# Autodesk Inventor assembly: ECE477
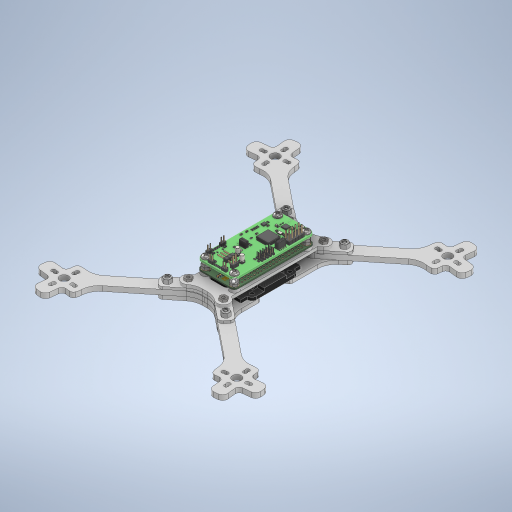
[picture p0: Inventor's stored thumbnail of the model, 512x512]
Saved by Autodesk Inventor 2023 (Build 270158000, 158)
## iProperties
Created: 2022-11-05
Part Number: ECE477
Document SubType Name: Assembly
Designer: mjlangfo
Author: mjlangfo
## Documents named in this file (9)
- \\nas01.itap.purdue.edu\puhome\desktop\mechanical\ECE477.iam
- \\nas01.itap.purdue.edu\puhome\desktop\mechanical\Source Two v0.1_import.ipt
- \\nas01.itap.purdue.edu\puhome\desktop\mechanical\Flight Controller Mount.ipt
- \\nas01.itap.purdue.edu\puhome\desktop\mechanical\RapberryPiZero.iam
- \\nas01.itap.purdue.edu\puhome\desktop\mechanical\Velox ESC.ipt
- \\nas01.itap.purdue.edu\puhome\desktop\mechanical\ECE477_PCB (1).iam
- \\nas01.itap.purdue.edu\puhome\My Documents\Inventor\Content Center Files\R2023\en-US\SS-ISO 4032\ISO 4032 - M2.5SS-ISO.ipt
- \\nas01.itap.purdue.edu\puhome\My Documents\Inventor\Content Center Files\R2023\en-US\AS 1427(08)\AS 1427 - M3 x 5(6) I.ipt
- \\nas01.itap.purdue.edu\puhome\My Documents\Inventor\Content Center Files\R2023\en-US\NF EN 24036\NF EN 24036 - M2.5.ipt
## Components (25 placed, 8 different names)
1. Source Two v0.1_import:1 — Flush:1, Flush:2
2. Flight Controller Mount:1 — Flush:1, Rotational:3, Rotational:4, Insert:17, Insert:18, Insert:19, Insert:20
3. RapberryPiZero:1 [sub-assembly] — Insert:1, Insert:4, Insert:7, Insert:10, Rotational:3, Rotational:4
4. Velox ESC:1 — Flush:2
5. ECE477_PCB (1):1 [sub-assembly] — Rotational:1, Rotational:2, Insert:13, Insert:14, Insert:15, Insert:16
6. SS ISO 4032 M2.5:1 — Insert:1, Insert:2
7. SS ISO 4032 M2.5:2 — Insert:2, Insert:3
8. SS ISO 4032 M2.5:3 — Insert:3
9. SS ISO 4032 M2.5:4 — Insert:4, Insert:5
10. SS ISO 4032 M2.5:5 — Insert:5, Insert:6
11. SS ISO 4032 M2.5:6 — Insert:6
12. SS ISO 4032 M2.5:7 — Insert:7, Insert:8
13. SS ISO 4032 M2.5:8 — Insert:8, Insert:9
14. SS ISO 4032 M2.5:9 — Insert:9, Rotational:1
15. SS ISO 4032 M2.5:10 — Insert:10, Insert:11
16. SS ISO 4032 M2.5:11 — Insert:11, Insert:12
17. SS ISO 4032 M2.5:12 — Insert:12, Rotational:2
18. AS 1427 Z - Metric M3 x 5:1 — Insert:13
19. AS 1427 Z - Metric M3 x 5:2 — Insert:14
20. AS 1427 Z - Metric M3 x 5:3 — Insert:15
21. AS 1427 Z - Metric M3 x 5:4 — Insert:16
22. NF EN 24036 M2.5:1 — Insert:17
23. NF EN 24036 M2.5:2 — Insert:18
24. NF EN 24036 M2.5:3 — Insert:19
25. NF EN 24036 M2.5:4 — Insert:20
## Relationships (26: Insert 20, RevoluteJoint 4, Flush 2)
- Flush:1: Source Two v0.1_import:1 ↔ Flight Controller Mount:1
- Flush:2: Source Two v0.1_import:1 ↔ Velox ESC:1
- Insert:1: RapberryPiZero:1 ↔ SS ISO 4032 M2.5:1
- Insert:2: SS ISO 4032 M2.5:1 ↔ SS ISO 4032 M2.5:2
- Insert:3: SS ISO 4032 M2.5:2 ↔ SS ISO 4032 M2.5:3
- Insert:4: RapberryPiZero:1 ↔ SS ISO 4032 M2.5:4
- Insert:5: SS ISO 4032 M2.5:4 ↔ SS ISO 4032 M2.5:5
- Insert:6: SS ISO 4032 M2.5:5 ↔ SS ISO 4032 M2.5:6
- Insert:7: RapberryPiZero:1 ↔ SS ISO 4032 M2.5:7
- Insert:8: SS ISO 4032 M2.5:7 ↔ SS ISO 4032 M2.5:8
- Insert:9: SS ISO 4032 M2.5:8 ↔ SS ISO 4032 M2.5:9
- Insert:10: RapberryPiZero:1 ↔ SS ISO 4032 M2.5:10
- Insert:11: SS ISO 4032 M2.5:10 ↔ SS ISO 4032 M2.5:11
- Insert:12: SS ISO 4032 M2.5:11 ↔ SS ISO 4032 M2.5:12
- Rotational:1 [RevoluteJoint]: ECE477_PCB (1):1 ↔ SS ISO 4032 M2.5:9
- Rotational:2 [RevoluteJoint]: ECE477_PCB (1):1 ↔ SS ISO 4032 M2.5:12
- Insert:13: ECE477_PCB (1):1 ↔ AS 1427 Z - Metric M3 x 5:1
- Insert:14: ECE477_PCB (1):1 ↔ AS 1427 Z - Metric M3 x 5:2
- Insert:15: ECE477_PCB (1):1 ↔ AS 1427 Z - Metric M3 x 5:3
- Insert:16: ECE477_PCB (1):1 ↔ AS 1427 Z - Metric M3 x 5:4
- Rotational:3 [RevoluteJoint]: Flight Controller Mount:1 ↔ RapberryPiZero:1
- Rotational:4 [RevoluteJoint]: Flight Controller Mount:1 ↔ RapberryPiZero:1
- Insert:17: Flight Controller Mount:1 ↔ NF EN 24036 M2.5:1
- Insert:18: Flight Controller Mount:1 ↔ NF EN 24036 M2.5:2
- Insert:19: Flight Controller Mount:1 ↔ NF EN 24036 M2.5:3
- Insert:20: Flight Controller Mount:1 ↔ NF EN 24036 M2.5:4
